# Autodesk Inventor assembly: J005233
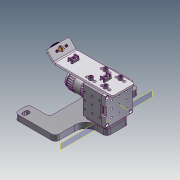
[picture p0: Inventor's stored thumbnail of the model, 180x180]
Saved by Autodesk Inventor 2015 SP1 (Build 190203100, 203)
## iProperties
Created: 2008-09-29
Part Number: J005233
Document SubType Name: Assembly
Designer: duttaa
Description: MBS CAMERA ASSY
Project: COMMON
Vendor: HHMI: JRC - ID&F
Translation Standard: STEP AP214IS
File Name: C:\Documents and Settings\duttaa\My Documents\Project Docus\6926\Camera Assembly.stp
Preprocessor: Autodesk Inventor 2008
Postprocessor: Build: 284, Release: 2008 SP1 - Date: Fri 07/06/2007
Sent Units: INCHES
Uncertainty: 0.00039370078740199997
ALTERED ITEM DESCRIPTION: N/A
ALTERED ITEM PART NUMBER: N/A
ALTERED ITEM VENDOR: N/A
DESIGN DEPARTMENT: HHMI: JRC - ID&F
LAB/DEPT: COMMON
REQUESTING SCIENTIST: COMMON
SPECIAL FINISH: NONE
SURFACE ROUGHNESS: N/A
Revision Number: 0
## Documents named in this file (19)
- C:\_WORKSPACE\DATA\COLLABORATION\SVOBODA LAB\MOUSE POSITIONING SYSTEMS\MCAD\BALL SETUP\MBS CAMERA ASSY.iam
- C:\_WORKSPACE\DATA\COLLABORATION\SVOBODA LAB\MOUSE POSITIONING SYSTEMS\MCAD\BALL SETUP\Camera Front body.ipt
- C:\_WORKSPACE\DATA\COLLABORATION\SVOBODA LAB\MOUSE POSITIONING SYSTEMS\MCAD\BALL SETUP\PCB.ipt
- C:\_WORKSPACE\DATA\COLLABORATION\SVOBODA LAB\MOUSE POSITIONING SYSTEMS\MCAD\BALL SETUP\Ribbon Cable Connector.ipt
- C:\_WORKSPACE\DATA\COLLABORATION\SVOBODA LAB\MOUSE POSITIONING SYSTEMS\MCAD\BALL SETUP\Camera Back Plate.ipt
- C:\_WORKSPACE\DATA\COLLABORATION\SVOBODA LAB\MOUSE POSITIONING SYSTEMS\MCAD\BALL SETUP\MBS C LED BRKT.ipt
- C:\_WORKSPACE\DATA\COLLABORATION\SVOBODA LAB\MOUSE POSITIONING SYSTEMS\MCAD\BALL SETUP\321527B00000G.ipt
- C:\_WORKSPACE\DATA\COLLABORATION\SVOBODA LAB\MOUSE POSITIONING SYSTEMS\MCAD\BALL SETUP\OD-110L.ipt
- C:\_WORKSPACE\DATA\COLLABORATION\SVOBODA LAB\MOUSE POSITIONING SYSTEMS\MCAD\BALL SETUP\TM1S4.ipt
- C:\_WORKSPACE\DATA\COLLABORATION\SVOBODA LAB\MOUSE POSITIONING SYSTEMS\MCAD\BALL SETUP\90116A147.ipt
- C:\_WORKSPACE\DATA\COLLABORATION\SVOBODA LAB\MOUSE POSITIONING SYSTEMS\MCAD\BALL SETUP\92196A190.ipt
- C:\_WORKSPACE\DATA\COLLABORATION\SVOBODA LAB\MOUSE POSITIONING SYSTEMS\MCAD\BALL SETUP\92196A077.ipt
- C:\_WORKSPACE\DATA\COLLABORATION\SVOBODA LAB\MOUSE POSITIONING SYSTEMS\MCAD\BALL SETUP\MBS Camera Spacer.ipt
- C:\_WORKSPACE\DATA\COLLABORATION\SVOBODA LAB\MOUSE POSITIONING SYSTEMS\MCAD\BALL SETUP\MBS Camera Bracket.ipt
- C:\_WORKSPACE\DATA\COLLABORATION\SVOBODA LAB\MOUSE POSITIONING SYSTEMS\MCAD\BALL SETUP\03-618.ipt
- C:\_WORKSPACE\DATA\COLLABORATION\SVOBODA LAB\MOUSE POSITIONING SYSTEMS\MCAD\BALL SETUP\M2514-MP2.ipt
- C:\_WORKSPACE\DATA\COLLABORATION\SVOBODA LAB\MOUSE POSITIONING SYSTEMS\MCAD\BALL SETUP\90107A010.ipt
- C:\_WORKSPACE\DATA\COLLABORATION\SVOBODA LAB\MOUSE POSITIONING SYSTEMS\MCAD\BALL SETUP\92196A198.ipt
- C:\_WORKSPACE\DATA\COLLABORATION\SVOBODA LAB\MOUSE POSITIONING SYSTEMS\MCAD\BALL SETUP\91772A110.ipt
## Components (31 placed, 18 different names)
1. Camera Front body:1 — Mate:1, Mate:2, Mate:3, Mate:14, Mate:16, Mate:18, Mate:20, Mate:39, Mate:40
2. MBS Camera Spacer:2 — Mate:44
3. MBS Camera Bracket:2 — Mate:43
4. PCB:1
5. Ribbon Cable Connector:1
6. Camera Back Plate:1
7. 91772A110:1
8. 91772A110:2
9. 91772A110:3
10. 91772A110:4
11. 91772A110:5
12. 91772A110:6
13. 91772A110:7
14. 91772A110:8
15. MBS C LED BRKT:1 — Mate:1, Mate:2, Mate:3, Mate:4, Mate:5, Mate:6, Mate:9, Mate:10, Mate:11, Mate:12, Angle:1, Angle:2, Mate:13, Mate:15, Mate:17, Mate:19, Mate:22, Mate:25, Mate:26, Mate:27, Mate:28
16. 321527B00000G:1 — Mate:4, Mate:5, Mate:6, Mate:7, Mate:8
17. OD-110L:1 — Mate:7, Mate:8
18. TM1S4:1 — Mate:9, Mate:12, Angle:1, Mate:23, Mate:24
19. TM1S4:2 — Mate:10, Mate:11, Angle:2, Mate:21
20. 90116A147:1 — Mate:21, Mate:22
21. 90116A147:2 — Mate:23, Mate:24
22. 92196A190:1 — Mate:13, Mate:14
23. 92196A190:2 — Mate:15, Mate:16
24. 92196A190:3 — Mate:19, Mate:20
25. 92196A190:4 — Mate:17, Mate:18
26. 92196A077:1 — Mate:27, Mate:28
27. 92196A077:2 — Mate:25, Mate:26
28. 03-618:1 — Mate:39, Mate:40, Mate:41, Mate:42
29. M2514-MP2:1 — Mate:41, Mate:42
30. 90107A010:1 — Mate:43, Mate:44, Mate:45, Mate:46
31. 92196A198:1 — Mate:45, Mate:46
## Relationships (44: Mate 41, Angle 3)
- Mate:1: Camera Front body:1 ↔ MBS C LED BRKT:1
- Mate:2: Camera Front body:1 ↔ MBS C LED BRKT:1
- Mate:3: Camera Front body:1 ↔ MBS C LED BRKT:1
- Mate:4: MBS C LED BRKT:1 ↔ 321527B00000G:1
- Mate:5: MBS C LED BRKT:1 ↔ 321527B00000G:1
- Mate:6: MBS C LED BRKT:1 ↔ 321527B00000G:1
- Mate:7: 321527B00000G:1 ↔ OD-110L:1
- Mate:8: 321527B00000G:1 ↔ OD-110L:1
- Mate:9: MBS C LED BRKT:1 ↔ TM1S4:1
- Mate:10: MBS C LED BRKT:1 ↔ TM1S4:2
- Mate:11: MBS C LED BRKT:1 ↔ TM1S4:2
- Mate:12: MBS C LED BRKT:1 ↔ TM1S4:1
- Angle:1 (0 deg): MBS C LED BRKT:1 ↔ TM1S4:1
- Angle:2 (0 deg): MBS C LED BRKT:1 ↔ TM1S4:2
- Mate:13: MBS C LED BRKT:1 ↔ 92196A190:1
- Mate:14: Camera Front body:1 ↔ 92196A190:1
- Mate:15: MBS C LED BRKT:1 ↔ 92196A190:2
- Mate:16: Camera Front body:1 ↔ 92196A190:2
- Mate:17: MBS C LED BRKT:1 ↔ 92196A190:4
- Mate:18: Camera Front body:1 ↔ 92196A190:4
- Mate:19: MBS C LED BRKT:1 ↔ 92196A190:3
- Mate:20: Camera Front body:1 ↔ 92196A190:3
- Mate:21: TM1S4:2 ↔ 90116A147:1
- Mate:22: MBS C LED BRKT:1 ↔ 90116A147:1
- Mate:23: TM1S4:1 ↔ 90116A147:2
- Mate:24: TM1S4:1 ↔ 90116A147:2
- Mate:25: MBS C LED BRKT:1 ↔ 92196A077:2
- Mate:26: MBS C LED BRKT:1 ↔ 92196A077:2
- Mate:27: MBS C LED BRKT:1 ↔ 92196A077:1
- Mate:28: MBS C LED BRKT:1 ↔ 92196A077:1
- [Mate] (6.35 mm): Camera Front body:1 ↔ MBS Camera Bracket:2
- [Mate]: Camera Front body:1 ↔ MBS Camera Bracket:2
- [Angle] (180 deg): MBS Camera Bracket:2
- [Mate]: MBS Camera Spacer:2 ↔ MBS Camera Bracket:2
- [Mate]: Camera Front body:1 ↔ MBS Camera Spacer:2
- [Mate]: Camera Front body:1 ↔ MBS Camera Spacer:2
- Mate:39: Camera Front body:1 ↔ 03-618:1
- Mate:40: Camera Front body:1 ↔ 03-618:1
- Mate:41: 03-618:1 ↔ M2514-MP2:1
- Mate:42: 03-618:1 ↔ M2514-MP2:1
- Mate:43: MBS Camera Bracket:2 ↔ 90107A010:1
- Mate:44: MBS Camera Spacer:2 ↔ 90107A010:1
- Mate:45: 90107A010:1 ↔ 92196A198:1
- Mate:46: 90107A010:1 ↔ 92196A198:1
